# Autodesk Inventor assembly: printer
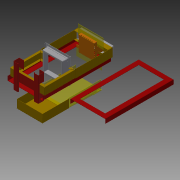
[picture p0: Inventor's stored thumbnail of the model, 180x180]
Saved by Autodesk Inventor 2014 SP2 (Build 180246200, 246)
## iProperties
Created: 2016-04-26
Part Number: printer
Document SubType Name: Assembly
Designer: cruiser
Author: cruiser
## Documents named in this file (11)
- C:\Users\cruiser\Desktop\models\3d printers\laserresin4\printer.iam
- C:\Users\cruiser\Desktop\models\3d printers\laserresin4\frame_inner.ipt
- C:\Users\cruiser\Desktop\models\3d printers\laserresin4\frame_face.ipt
- C:\Users\cruiser\Desktop\models\3d printers\laserresin4\crane.ipt
- C:\Users\cruiser\Desktop\models\3d printers\laserresin4\bed.ipt
- C:\Users\cruiser\Desktop\models\3d printers\laserresin4\carrier.ipt
- C:\Users\cruiser\Desktop\models\3d printers\laserresin4\reservoir.ipt
- C:\Users\cruiser\Desktop\models\3d printers\laserresin4\frame_feet.ipt
- C:\Users\cruiser\Desktop\models\3d printers\laserresin4\frame_lower.ipt
- C:\Users\cruiser\Desktop\models\3d printers\laserresin4\visor.ipt
- C:\Users\cruiser\Desktop\models\3d printers\laserresin4\door_assembly.iam
## Components (12 placed, 10 different names)
1. frame_inner:1 — Mate:2, Mate:3, Mate:6, Mate:12, Mate:13
2. frame_face:1
3. frame_face:2 — Mate:15
4. crane:1 — Mate:1, Mate:4, Mate:5
5. bed:1 — Mate:1
6. carrier:1 — Mate:2, Mate:3, Mate:4, Mate:5, Mate:6, Flush:1, Mate:7, Mate:8, Mate:9
7. reservoir:1 — Flush:1
8. frame_feet:1 — Mate:10, Mate:14
9. frame_lower:1 — Mate:7, Mate:8, Mate:9, Mate:10
10. visor:1 — Mate:12
11. visor:2 — Mate:13
12. door_assembly:1 [sub-assembly] — Mate:14, Mate:15
## Relationships (15: Mate 14, Flush 1)
- Mate:1: crane:1 ↔ bed:1
- Mate:2: frame_inner:1 ↔ carrier:1
- Mate:3: frame_inner:1 ↔ carrier:1
- Mate:4: crane:1 ↔ carrier:1
- Mate:5: crane:1 ↔ carrier:1
- Mate:6: frame_inner:1 ↔ carrier:1
- Flush:1: carrier:1 ↔ reservoir:1
- Mate:7: carrier:1 ↔ frame_lower:1
- Mate:8: carrier:1 ↔ frame_lower:1
- Mate:9: carrier:1 ↔ frame_lower:1
- Mate:10: frame_feet:1 ↔ frame_lower:1
- Mate:12: frame_inner:1 ↔ visor:1
- Mate:13: frame_inner:1 ↔ visor:2
- Mate:14: frame_feet:1 ↔ door_assembly:1
- Mate:15: frame_face:2 ↔ door_assembly:1
